# Autodesk Inventor assembly: nc_nhk26
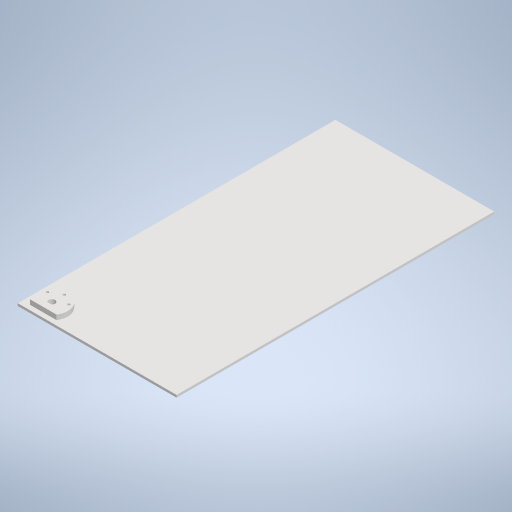
[picture p0: Inventor's stored thumbnail of the model, 512x512]
Saved by Autodesk Inventor 2023 (Build 270158000, 158)
## iProperties
Created: 2022-05-04
Part Number: nc_nhk26
Document SubType Name: Assembly
Designer: yuta
Author: yuta
## Documents named in this file (3)
- C:\Users\yuta\Documents\NHK\nc_nhk26.iam
- C:\Users\yuta\Documents\NHK\NC.port.ipt
- C:\Users\yuta\Documents\NHK\射出_留め具2.ipt
## Components (2 placed, 2 different names)
1. NC.port:1 — メイト:1, フラッシュ:1, メイト:2
2. 射出_留め具2:1 — メイト:1, フラッシュ:1, メイト:2
## Relationships (3: Mate 2, Flush 1)
- メイト:1 [Mate]: NC.port:1 ↔ 射出_留め具2:1
- フラッシュ:1 [Flush] (6 mm): NC.port:1 ↔ 射出_留め具2:1
- メイト:2 [Mate] (-26 mm): NC.port:1 ↔ 射出_留め具2:1
